# Autodesk Inventor assembly: final
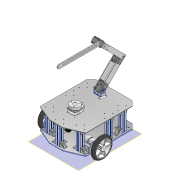
[picture p0: Inventor's stored thumbnail of the model, 180x180]
Saved by Autodesk Inventor 2020 (Build 240168000, 168)
## iProperties
Created: 2020-09-06
Part Number: final
Document SubType Name: Assembly
Designer: 이호석
Mass: 7439.99 g
Surface Area: 16173.7 cm^2
Volume: 3301.42 cm^3
Density: 2.25358 g/cm^3
Author: 이호석
## Documents named in this file (13)
- C:\Inventor\Embedded_contest\new_mobile\final.iam
- C:\Inventor\Embedded_contest\new_mobile\bottom.ipt
- C:\Inventor\Embedded_contest\new_mobile\top.ipt
- C:\Inventor\Embedded_contest\motor_support2.ipt
- C:\Inventor\Embedded_contest\ig42gm\IG-42GM+Encoder(49ratio).iam
- C:\Inventor\Embedded_contest\castor\castor_1inch.iam
- C:\Inventor\Embedded_contest\LIDAR\RPLIDAR_A1.iam
- C:\Inventor\Embedded_contest\new_mobile\motor_wall.ipt
- C:\Inventor\Embedded_contest\new_mobile\profile.ipt
- C:\Inventor\Embedded_contest\new_mobile\braket2.ipt
- C:\Inventor\Embedded_contest\145pi_wheel\145pi_tire.iam
- C:\Inventor\Embedded_contest\robotarm\robotarm.iam
- C:\Inventor\Embedded_contest\new_mobile\support.ipt
## Components (67 placed, 12 different names)
1. bottom:1 — 메이트:1, 플러쉬:1, 플러쉬:2, 플러쉬:3, 메이트:2, 메이트:3, 플러쉬:4, 플러쉬:6, 메이트:8, 메이트:9, 메이트:10, 메이트:11, 메이트:12, 메이트:13, 플러쉬:10, 플러쉬:11, 플러쉬:12, 플러쉬:13, 플러쉬:14, 플러쉬:15, 플러쉬:16, 플러쉬:17, 메이트:14, 메이트:15, 플러쉬:18, 플러쉬:19, 메이트:18, 플러쉬:20, 플러쉬:21, 메이트:19, 메이트:21, 메이트:23, 메이트:25, 메이트:27, 메이트:29, 메이트:31, 메이트:32, 메이트:33, 메이트:37, 메이트:38, 메이트:39, 메이트:43, 메이트:44, 메이트:45, 메이트:49, 메이트:50, 메이트:51, 메이트:55, 메이트:56, 메이트:57, 메이트:61, 메이트:62, 메이트:65, 메이트:66, 플러쉬:68, 삽입:28, 삽입:29, 삽입:30, 삽입:31
2. top:1 — 메이트:1, 플러쉬:1, 플러쉬:2, 삽입:13, 삽입:14, 삽입:15, 삽입:16, 메이트:69, 메이트:70, 메이트:71, 메이트:75, 메이트:76, 메이트:77, 메이트:81, 메이트:82, 메이트:83, 메이트:87, 메이트:88, 메이트:89, 메이트:93, 메이트:94, 메이트:95, 메이트:99, 메이트:100, 메이트:101, 메이트:105, 메이트:106, 메이트:107, 메이트:111, 메이트:112, 플러쉬:69
3. RPLIDAR_A1:1 [sub-assembly] — 삽입:13, 삽입:14, 삽입:15, 삽입:16
4. robotarm:1 [sub-assembly] — 메이트:111, 메이트:112, 플러쉬:69
5. motor_support2:1 — 플러쉬:3, 메이트:2, 플러쉬:5, 플러쉬:6, 삽입:2
6. motor_support2:2 — 메이트:3, 플러쉬:4, 플러쉬:5, 삽입:1
7. IG-42GM+Encoder(49ratio):1 [sub-assembly] — 삽입:1, 삽입:22, 삽입:23, 삽입:24, 삽입:25, 삽입:33
8. IG-42GM+Encoder(49ratio):2 [sub-assembly] — 삽입:2, 삽입:17, 삽입:18, 삽입:19, 삽입:20, 삽입:21, 삽입:32
9. 145pi_tire:1 [sub-assembly] — 삽입:33
10. 145pi_tire:2 [sub-assembly] — 삽입:32
11. castor_1inch:1 [sub-assembly] — 삽입:28, 삽입:29, 삽입:30, 삽입:31, 플러쉬:70
12. support:1 — 플러쉬:70
13. motor_wall:1 — 메이트:8, 삽입:22, 삽입:23, 삽입:24, 삽입:25, 메이트:67, 메이트:68, 플러쉬:45, 플러쉬:46
14. motor_wall:2 — 메이트:9, 삽입:17, 삽입:18, 삽입:19, 삽입:20, 삽입:21, 메이트:63, 메이트:64, 플러쉬:43, 플러쉬:44
15. profile:1 — 메이트:12, 플러쉬:11, 플러쉬:16, 메이트:26, 플러쉬:25, 메이트:28, 플러쉬:26, 메이트:30, 플러쉬:27, 메이트:78, 메이트:79, 메이트:80, 플러쉬:50, 플러쉬:51, 플러쉬:52
16. profile:2 — 메이트:11, 플러쉬:12, 플러쉬:17, 메이트:34, 메이트:35, 메이트:36, 플러쉬:28, 플러쉬:29, 플러쉬:30, 메이트:84, 메이트:85, 메이트:86, 플러쉬:53, 플러쉬:54, 플러쉬:55
17. profile:3 — 메이트:10, 플러쉬:10, 플러쉬:15, 메이트:16, 메이트:52, 메이트:53, 메이트:54, 플러쉬:37, 플러쉬:38, 플러쉬:39, 메이트:108, 메이트:109, 메이트:110, 플러쉬:65, 플러쉬:66, 플러쉬:67
18. profile:4 — 메이트:13, 플러쉬:13, 플러쉬:14, 메이트:17, 메이트:58, 메이트:59, 메이트:60, 플러쉬:40, 플러쉬:41, 플러쉬:42, 메이트:102, 메이트:103, 메이트:104, 플러쉬:62, 플러쉬:63, 플러쉬:64
19. profile:5 — 메이트:15, 플러쉬:19, 메이트:16, 메이트:40, 메이트:41, 메이트:42, 플러쉬:31, 플러쉬:32, 플러쉬:33, 메이트:96, 메이트:97, 메이트:98, 플러쉬:59, 플러쉬:60, 플러쉬:61
20. profile:6 — 메이트:14, 플러쉬:18, 메이트:17, 메이트:46, 메이트:47, 메이트:48, 플러쉬:34, 플러쉬:35, 플러쉬:36, 메이트:90, 메이트:91, 메이트:92, 플러쉬:56, 플러쉬:57, 플러쉬:58
21. profile:7 — 메이트:18, 플러쉬:20, 플러쉬:21, 메이트:20, 플러쉬:22, 메이트:22, 플러쉬:23, 메이트:24, 플러쉬:24, 메이트:72, 메이트:73, 메이트:74, 플러쉬:47, 플러쉬:48, 플러쉬:49
22. braket2:1 — 메이트:19, 메이트:20, 플러쉬:22
23. braket2:2 — 메이트:21, 메이트:22, 플러쉬:23
24. braket2:3 — 메이트:23, 메이트:24, 플러쉬:24
25. braket2:4 — 메이트:25, 메이트:26, 플러쉬:25
26. braket2:5 — 메이트:27, 메이트:28, 플러쉬:26
27. braket2:6 — 메이트:29, 메이트:30, 플러쉬:27
28. braket2:7 — 메이트:32, 메이트:34, 플러쉬:30
29. braket2:8 — 메이트:31, 메이트:36, 플러쉬:28
30. braket2:9 — 메이트:33, 메이트:35, 플러쉬:29
31. braket2:10 — 메이트:37, 메이트:42, 플러쉬:32
32. braket2:11 — 메이트:38, 메이트:41, 플러쉬:33
33. braket2:12 — 메이트:39, 메이트:40, 플러쉬:31
34. braket2:13 — 메이트:43, 메이트:46, 플러쉬:36
35. braket2:14 — 메이트:44, 메이트:48, 플러쉬:35
36. braket2:15 — 메이트:45, 메이트:47, 플러쉬:34
37. braket2:16 — 메이트:51, 메이트:52, 플러쉬:38
38. braket2:17 — 메이트:50, 메이트:54, 플러쉬:37
39. braket2:18 — 메이트:49, 메이트:53, 플러쉬:39
40. braket2:19 — 메이트:55, 메이트:59, 플러쉬:42
41. braket2:20 — 메이트:57, 메이트:60, 플러쉬:40
42. braket2:21 — 메이트:56, 메이트:58, 플러쉬:41
43. braket2:26 — 메이트:69, 메이트:73, 플러쉬:48
44. braket2:27 — 메이트:70, 메이트:74, 플러쉬:47
45. braket2:28 — 메이트:71, 메이트:72, 플러쉬:49
46. braket2:29 — 메이트:77, 메이트:80, 플러쉬:50
47. braket2:30 — 메이트:76, 메이트:79, 플러쉬:51
48. braket2:31 — 메이트:75, 메이트:78, 플러쉬:52
49. braket2:32 — 메이트:81, 메이트:84, 플러쉬:55
50. braket2:33 — 메이트:82, 메이트:85, 플러쉬:53
51. braket2:34 — 메이트:83, 메이트:86, 플러쉬:54
52. braket2:35 — 메이트:87, 메이트:92, 플러쉬:56
53. braket2:36 — 메이트:88, 메이트:90, 플러쉬:57
54. braket2:37 — 메이트:89, 메이트:91, 플러쉬:58
55. braket2:38 — 메이트:93, 메이트:98, 플러쉬:59
56. braket2:39 — 메이트:94, 메이트:97, 플러쉬:60
57. braket2:40 — 메이트:95, 메이트:96, 플러쉬:61
58. braket2:41 — 메이트:99, 메이트:102, 플러쉬:64
59. braket2:42 — 메이트:100, 메이트:104, 플러쉬:63
60. braket2:43 — 메이트:101, 메이트:103, 플러쉬:62
61. braket2:44 — 메이트:105, 메이트:110, 플러쉬:65
62. braket2:45 — 메이트:106, 메이트:109, 플러쉬:66
63. braket2:46 — 메이트:107, 메이트:108, 플러쉬:67
64. braket2:22 — 메이트:61, 메이트:64, 플러쉬:43
65. braket2:23 — 메이트:62, 메이트:63, 플러쉬:44
66. braket2:24 — 메이트:65, 메이트:68, 플러쉬:45
67. braket2:25 — 메이트:66, 메이트:67, 플러쉬:46
## Relationships (196: Mate 108, Flush 67, Insert 21)
- 메이트:1 [Mate] (144.5 mm): bottom:1 ↔ top:1
- 플러쉬:1 [Flush]: bottom:1 ↔ top:1
- 플러쉬:2 [Flush]: bottom:1 ↔ top:1
- 플러쉬:3 [Flush] (5 mm): bottom:1 ↔ motor_support2:1
- 메이트:2 [Mate]: bottom:1 ↔ motor_support2:1
- 메이트:3 [Mate]: bottom:1 ↔ motor_support2:2
- 플러쉬:4 [Flush] (5 mm): bottom:1 ↔ motor_support2:2
- 플러쉬:5 [Flush]: motor_support2:1 ↔ motor_support2:2
- 플러쉬:6 [Flush] (115 mm): bottom:1 ↔ motor_support2:1
- 삽입:1 [Insert]: motor_support2:2 ↔ IG-42GM+Encoder(49ratio):1
- 삽입:2 [Insert]: motor_support2:1 ↔ IG-42GM+Encoder(49ratio):2
- 삽입:13 [Insert]: top:1 ↔ RPLIDAR_A1:1
- 삽입:14 [Insert]: top:1 ↔ RPLIDAR_A1:1
- 삽입:15 [Insert]: top:1 ↔ RPLIDAR_A1:1
- 삽입:16 [Insert]: top:1 ↔ RPLIDAR_A1:1
- 메이트:8 [Mate]: bottom:1 ↔ motor_wall:1
- 메이트:9 [Mate]: bottom:1 ↔ motor_wall:2
- 삽입:17 [Insert]: IG-42GM+Encoder(49ratio):2 ↔ motor_wall:2
- 삽입:18 [Insert]: IG-42GM+Encoder(49ratio):2 ↔ motor_wall:2
- 삽입:19 [Insert]: IG-42GM+Encoder(49ratio):2 ↔ motor_wall:2
- 삽입:20 [Insert]: IG-42GM+Encoder(49ratio):2 ↔ motor_wall:2
- 삽입:21 [Insert]: IG-42GM+Encoder(49ratio):2 ↔ motor_wall:2
- 삽입:22 [Insert]: IG-42GM+Encoder(49ratio):1 ↔ motor_wall:1
- 삽입:23 [Insert]: IG-42GM+Encoder(49ratio):1 ↔ motor_wall:1
- 삽입:24 [Insert]: IG-42GM+Encoder(49ratio):1 ↔ motor_wall:1
- 삽입:25 [Insert]: IG-42GM+Encoder(49ratio):1 ↔ motor_wall:1
- 메이트:10 [Mate]: bottom:1 ↔ profile:3
- 메이트:11 [Mate]: bottom:1 ↔ profile:2
- 메이트:12 [Mate]: bottom:1 ↔ profile:1
- 메이트:13 [Mate]: bottom:1 ↔ profile:4
- 플러쉬:10 [Flush] (10 mm): bottom:1 ↔ profile:3
- 플러쉬:11 [Flush] (40 mm): bottom:1 ↔ profile:1
- 플러쉬:12 [Flush] (-40 mm): bottom:1 ↔ profile:2
- 플러쉬:13 [Flush] (10 mm): bottom:1 ↔ profile:4
- 플러쉬:14 [Flush] (-70 mm): bottom:1 ↔ profile:4
- 플러쉬:15 [Flush] (70 mm): bottom:1 ↔ profile:3
- 플러쉬:16 [Flush] (-50 mm): bottom:1 ↔ profile:1
- 플러쉬:17 [Flush] (-50 mm): bottom:1 ↔ profile:2
- 메이트:14 [Mate]: bottom:1 ↔ profile:6
- 메이트:15 [Mate]: bottom:1 ↔ profile:5
- 플러쉬:18 [Flush] (10 mm): bottom:1 ↔ profile:6
- 플러쉬:19 [Flush] (10 mm): bottom:1 ↔ profile:5
- 메이트:16 [Mate] (70 mm): profile:3 ↔ profile:5
- 메이트:17 [Mate] (70 mm): profile:4 ↔ profile:6
- 메이트:18 [Mate]: bottom:1 ↔ profile:7
- 플러쉬:20 [Flush] (10 mm): bottom:1 ↔ profile:7
- 플러쉬:21 [Flush] (155 mm): bottom:1 ↔ profile:7
- 메이트:19 [Mate]: bottom:1 ↔ braket2:1
- 메이트:20 [Mate]: profile:7 ↔ braket2:1
- 플러쉬:22 [Flush] (2.5 mm): profile:7 ↔ braket2:1
- 메이트:21 [Mate]: bottom:1 ↔ braket2:2
- 메이트:22 [Mate]: profile:7 ↔ braket2:2
- 플러쉬:23 [Flush] (2.5 mm): profile:7 ↔ braket2:2
- 메이트:23 [Mate]: bottom:1 ↔ braket2:3
- 메이트:24 [Mate]: profile:7 ↔ braket2:3
- 플러쉬:24 [Flush] (2.5 mm): profile:7 ↔ braket2:3
- 메이트:25 [Mate]: bottom:1 ↔ braket2:4
- 메이트:26 [Mate]: profile:1 ↔ braket2:4
- 플러쉬:25 [Flush] (2.5 mm): profile:1 ↔ braket2:4
- 메이트:27 [Mate]: bottom:1 ↔ braket2:5
- 메이트:28 [Mate]: profile:1 ↔ braket2:5
- 플러쉬:26 [Flush] (2.5 mm): profile:1 ↔ braket2:5
- 메이트:29 [Mate]: bottom:1 ↔ braket2:6
- 메이트:30 [Mate]: profile:1 ↔ braket2:6
- 플러쉬:27 [Flush] (2.5 mm): profile:1 ↔ braket2:6
- 메이트:31 [Mate]: bottom:1 ↔ braket2:8
- 메이트:32 [Mate]: bottom:1 ↔ braket2:7
- 메이트:33 [Mate]: bottom:1 ↔ braket2:9
- 메이트:34 [Mate]: profile:2 ↔ braket2:7
- 메이트:35 [Mate]: profile:2 ↔ braket2:9
- 메이트:36 [Mate]: profile:2 ↔ braket2:8
- 플러쉬:28 [Flush] (2.5 mm): profile:2 ↔ braket2:8
- 플러쉬:29 [Flush] (2.5 mm): profile:2 ↔ braket2:9
- 플러쉬:30 [Flush] (2.5 mm): profile:2 ↔ braket2:7
- 메이트:37 [Mate]: bottom:1 ↔ braket2:10
- 메이트:38 [Mate]: bottom:1 ↔ braket2:11
- 메이트:39 [Mate]: bottom:1 ↔ braket2:12
- 메이트:40 [Mate]: profile:5 ↔ braket2:12
- 메이트:41 [Mate]: profile:5 ↔ braket2:11
- 메이트:42 [Mate]: profile:5 ↔ braket2:10
- 플러쉬:31 [Flush] (2.5 mm): profile:5 ↔ braket2:12
- 플러쉬:32 [Flush] (2.5 mm): profile:5 ↔ braket2:10
- 플러쉬:33 [Flush] (2.5 mm): profile:5 ↔ braket2:11
- 메이트:43 [Mate]: bottom:1 ↔ braket2:13
- 메이트:44 [Mate]: bottom:1 ↔ braket2:14
- 메이트:45 [Mate]: bottom:1 ↔ braket2:15
- 메이트:46 [Mate]: profile:6 ↔ braket2:13
- 메이트:47 [Mate]: profile:6 ↔ braket2:15
- 메이트:48 [Mate]: profile:6 ↔ braket2:14
- 플러쉬:34 [Flush] (2.5 mm): profile:6 ↔ braket2:15
- 플러쉬:35 [Flush] (2.5 mm): profile:6 ↔ braket2:14
- 플러쉬:36 [Flush] (2.5 mm): profile:6 ↔ braket2:13
- 메이트:49 [Mate]: bottom:1 ↔ braket2:18
- 메이트:50 [Mate]: bottom:1 ↔ braket2:17
- 메이트:51 [Mate]: bottom:1 ↔ braket2:16
- 메이트:52 [Mate]: profile:3 ↔ braket2:16
- 메이트:53 [Mate]: profile:3 ↔ braket2:18
- 메이트:54 [Mate]: profile:3 ↔ braket2:17
- 플러쉬:37 [Flush] (2.5 mm): profile:3 ↔ braket2:17
- 플러쉬:38 [Flush] (2.5 mm): profile:3 ↔ braket2:16
- 플러쉬:39 [Flush] (2.5 mm): profile:3 ↔ braket2:18
- 메이트:55 [Mate]: bottom:1 ↔ braket2:19
- 메이트:56 [Mate]: bottom:1 ↔ braket2:21
- 메이트:57 [Mate]: bottom:1 ↔ braket2:20
- 메이트:58 [Mate]: profile:4 ↔ braket2:21
- 메이트:59 [Mate]: profile:4 ↔ braket2:19
- 메이트:60 [Mate]: profile:4 ↔ braket2:20
- 플러쉬:40 [Flush] (2.5 mm): profile:4 ↔ braket2:20
- 플러쉬:41 [Flush] (2.5 mm): profile:4 ↔ braket2:21
- 플러쉬:42 [Flush] (2.5 mm): profile:4 ↔ braket2:19
- 메이트:61 [Mate]: bottom:1 ↔ braket2:22
- 메이트:62 [Mate]: bottom:1 ↔ braket2:23
- 메이트:63 [Mate]: motor_wall:2 ↔ braket2:23
- 메이트:64 [Mate]: motor_wall:2 ↔ braket2:22
- 플러쉬:43 [Flush] (7.5 mm): motor_wall:2 ↔ braket2:22
- 플러쉬:44 [Flush] (7.5 mm): motor_wall:2 ↔ braket2:23
- 메이트:65 [Mate]: bottom:1 ↔ braket2:24
- 메이트:66 [Mate]: bottom:1 ↔ braket2:25
- 메이트:67 [Mate]: motor_wall:1 ↔ braket2:25
- 메이트:68 [Mate]: motor_wall:1 ↔ braket2:24
- 플러쉬:45 [Flush] (7.5 mm): motor_wall:1 ↔ braket2:24
- 플러쉬:46 [Flush] (7.5 mm): motor_wall:1 ↔ braket2:25
- 메이트:69 [Mate]: top:1 ↔ braket2:26
- 메이트:70 [Mate]: top:1 ↔ braket2:27
- 메이트:71 [Mate]: top:1 ↔ braket2:28
- 메이트:72 [Mate]: profile:7 ↔ braket2:28
- 메이트:73 [Mate]: profile:7 ↔ braket2:26
- 메이트:74 [Mate]: profile:7 ↔ braket2:27
- 플러쉬:47 [Flush] (2.5 mm): profile:7 ↔ braket2:27
- 플러쉬:48 [Flush] (2.5 mm): profile:7 ↔ braket2:26
- 플러쉬:49 [Flush] (2.5 mm): profile:7 ↔ braket2:28
- 메이트:75 [Mate]: top:1 ↔ braket2:31
- 메이트:76 [Mate]: top:1 ↔ braket2:30
- 메이트:77 [Mate]: top:1 ↔ braket2:29
- 메이트:78 [Mate]: profile:1 ↔ braket2:31
- 메이트:79 [Mate]: profile:1 ↔ braket2:30
- 메이트:80 [Mate]: profile:1 ↔ braket2:29
- 플러쉬:50 [Flush] (2.5 mm): profile:1 ↔ braket2:29
- 플러쉬:51 [Flush] (2.5 mm): profile:1 ↔ braket2:30
- 플러쉬:52 [Flush] (2.5 mm): profile:1 ↔ braket2:31
- 메이트:81 [Mate]: top:1 ↔ braket2:32
- 메이트:82 [Mate]: top:1 ↔ braket2:33
- 메이트:83 [Mate]: top:1 ↔ braket2:34
- 메이트:84 [Mate]: profile:2 ↔ braket2:32
- 메이트:85 [Mate]: profile:2 ↔ braket2:33
- 메이트:86 [Mate]: profile:2 ↔ braket2:34
- 플러쉬:53 [Flush] (2.5 mm): profile:2 ↔ braket2:33
- 플러쉬:54 [Flush] (2.5 mm): profile:2 ↔ braket2:34
- 플러쉬:55 [Flush] (2.5 mm): profile:2 ↔ braket2:32
- 메이트:87 [Mate]: top:1 ↔ braket2:35
- 메이트:88 [Mate]: top:1 ↔ braket2:36
- 메이트:89 [Mate]: top:1 ↔ braket2:37
- 메이트:90 [Mate]: profile:6 ↔ braket2:36
- 메이트:91 [Mate]: profile:6 ↔ braket2:37
- 메이트:92 [Mate]: profile:6 ↔ braket2:35
- 플러쉬:56 [Flush] (2.5 mm): profile:6 ↔ braket2:35
- 플러쉬:57 [Flush] (2.5 mm): profile:6 ↔ braket2:36
- 플러쉬:58 [Flush] (2.5 mm): profile:6 ↔ braket2:37
- 메이트:93 [Mate]: top:1 ↔ braket2:38
- 메이트:94 [Mate]: top:1 ↔ braket2:39
- 메이트:95 [Mate]: top:1 ↔ braket2:40
- 메이트:96 [Mate]: profile:5 ↔ braket2:40
- 메이트:97 [Mate]: profile:5 ↔ braket2:39
- 메이트:98 [Mate]: profile:5 ↔ braket2:38
- 플러쉬:59 [Flush] (2.5 mm): profile:5 ↔ braket2:38
- 플러쉬:60 [Flush] (2.5 mm): profile:5 ↔ braket2:39
- 플러쉬:61 [Flush] (2.5 mm): profile:5 ↔ braket2:40
- 메이트:99 [Mate]: top:1 ↔ braket2:41
- 메이트:100 [Mate]: top:1 ↔ braket2:42
- 메이트:101 [Mate]: top:1 ↔ braket2:43
- 메이트:102 [Mate]: profile:4 ↔ braket2:41
- 메이트:103 [Mate]: profile:4 ↔ braket2:43
- 메이트:104 [Mate]: profile:4 ↔ braket2:42
- 플러쉬:62 [Flush] (2.5 mm): profile:4 ↔ braket2:43
- 플러쉬:63 [Flush] (2.5 mm): profile:4 ↔ braket2:42
- 플러쉬:64 [Flush] (2.5 mm): profile:4 ↔ braket2:41
- 메이트:105 [Mate]: top:1 ↔ braket2:44
- 메이트:106 [Mate]: top:1 ↔ braket2:45
- 메이트:107 [Mate]: top:1 ↔ braket2:46
- 메이트:108 [Mate]: profile:3 ↔ braket2:46
- 메이트:109 [Mate]: profile:3 ↔ braket2:45
- 메이트:110 [Mate]: profile:3 ↔ braket2:44
- 플러쉬:65 [Flush] (2.5 mm): profile:3 ↔ braket2:44
- 플러쉬:66 [Flush] (2.5 mm): profile:3 ↔ braket2:45
- 플러쉬:67 [Flush] (2.5 mm): profile:3 ↔ braket2:46
- 플러쉬:68 [Flush] (47.5 mm): bottom:1
- 삽입:28 [Insert] (12.5 mm): bottom:1 ↔ castor_1inch:1
- 삽입:29 [Insert] (12.5 mm): bottom:1 ↔ castor_1inch:1
- 삽입:30 [Insert] (12.5 mm): bottom:1 ↔ castor_1inch:1
- 삽입:31 [Insert] (12.5 mm): bottom:1 ↔ castor_1inch:1
- 삽입:32 [Insert] (-5 mm): IG-42GM+Encoder(49ratio):2 ↔ 145pi_tire:2
- 삽입:33 [Insert] (-5 mm): IG-42GM+Encoder(49ratio):1 ↔ 145pi_tire:1
- 메이트:111 [Mate]: top:1 ↔ robotarm:1
- 메이트:112 [Mate]: top:1 ↔ robotarm:1
- 플러쉬:69 [Flush] (10.1 mm): top:1 ↔ robotarm:1
- 플러쉬:70 [Flush]: castor_1inch:1 ↔ support:1
